# Autodesk Inventor assembly: Joint2
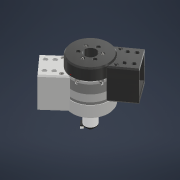
[picture p0: Inventor's stored thumbnail of the model, 180x180]
Saved by Autodesk Inventor 2021 (Build 250183000, 183)
## iProperties
RuleStatus: InUse
Created: 2025-03-14
Part Number: Joint2
Document SubType Name: Assembly
Designer: rocke
Mass: 414.793 g
Surface Area: 1158.92 cm^2
Volume: 253.092 cm^3
Density: 1.6389 g/cm^3
Author: rocke
## Documents named in this file (26)
- C:\Users\rocke\Documents\Robot Arm IPT\Joint2.iam
- C:\Users\rocke\Documents\Robot Arm IPT\Joint2\Design Accelerator\Spur Gears1.iam
- C:\Users\rocke\Documents\Robot Arm IPT\Joint2\Design Accelerator\Spur Gears3.iam
- C:\Users\rocke\Documents\Inventor\Content Center Files\R2021\en-US\DIN 472(2)\DIN 472 - 16x1.ipt
- C:\Users\rocke\Documents\Inventor\Content Center Files\R2021\en-US\DIN 625 SKF(4)\DIN 625 SKF - SKF 628_8-2Z.ipt
- C:\Users\rocke\Downloads\12V 350RPM Small DFRobot Motor v8.iam
- C:\Users\rocke\Documents\Inventor\Content Center Files\R2021\en-US\ISO 4762(2)\ISO 4762 - M3 x 5ISO.ipt
- C:\Users\rocke\Documents\Robot Arm IPT\Joint2\Design Accelerator\Spur Gear11.ipt
- C:\Users\rocke\Documents\Inventor\Content Center Files\R2021\en-US\GB_T 276-94 60000-2Z\Bearing 61809-2Z GB_T 276-94.ipt
- C:\Users\rocke\Documents\Robot Arm IPT\Joint2\Planet Subassembly.iam
- C:\Users\rocke\Downloads\TO-92 flat Formed Leads Horizontal Back.ipt
- C:\Users\rocke\Documents\Inventor\Content Center Files\R2021\en-US\ANSI B 18.2.4.1 M(1)\ANSI B 18.2.4.1 M - M3 x 0.5Style 1.ipt
- C:\Users\rocke\Documents\Inventor\Content Center Files\R2021\en-US\ISO 4026\ISO 4026 - M3 x 8 - ISO.ipt
- C:\Users\rocke\Documents\Inventor\Content Center Files\R2021\en-US\ANSI B18.3.1M(1)\ANSI B18.3.1M - M3x0.5 x 60(2).ipt
- C:\Users\rocke\Documents\Inventor\Content Center Files\R2021\en-US\DIN 985\DIN 985 - M3.ipt
- C:\Users\rocke\Documents\Inventor\Content Center Files\R2021\en-US\ISO 4032(2)\ISO 4032 - M4 - ISO.ipt
- C:\Users\rocke\Documents\Inventor\Content Center Files\R2021\en-US\ANSI B18.3.1M(1)\ANSI B18.3.1M - M4x0.7 x 60(2).ipt
- C:\Users\rocke\Documents\Inventor\Content Center Files\R2021\en-US\ANSI B18.3.1M(1)\ANSI B18.3.1M - M4x0.7 x 65(2).ipt
- C:\Users\rocke\Documents\Robot Arm IPT\Moving Link Fixation\Moving_Link_Fixation.iam
- C:\Users\rocke\Documents\Robot Arm IPT\Fixed Link Fixation\Fixed_Link_Fixation.iam
- C:\Users\rocke\Documents\Robot Arm IPT\Ring Gear 1\Ring_Gear_Assembly_1.iam
- C:\Users\rocke\Documents\Robot Arm IPT\Planet Carrier\Planet_Carrier_Bottom.ipt
- C:\Users\rocke\Documents\Robot Arm IPT\Planet Carrier\Planet_Carrier_Mid.ipt
- C:\Users\rocke\Documents\Robot Arm IPT\Planet Carrier\Planet_Carrier_Top.ipt
- C:\Users\rocke\Documents\Robot Arm IPT\Ring Cover\Ring_Cover_Bot.ipt
- C:\Users\rocke\Documents\Robot Arm IPT\Ring Cover\Ring_Cover_Top.ipt
## Components (44 placed, 24 different names)
1. Spur Gears:1 [sub-assembly]
2. Spur Gears:2 [sub-assembly] — Rigid:9, Rigid:13, Mate:16
3. Planet_Carrier_Bottom:1 — Rotational:3, Rotational:4, Rotational:5, Rigid:2, Rigid:4
4. Planet_Carrier_Mid:1 — Rigid:4, Rigid:5, Rigid:8
5. Planet_Carrier_Top:1 — Rigid:5, Rigid:7, Rigid:15
6. Ring_Cover_Bot:1 — Rotational:1, Mate:1, Mate:2, Mate:3, Mate:4, Mate:5, Rigid:9, Insert:2
7. Sun_Gear — Rotational:2, Rigid:1, Insert:1
8. Ring_Cover_Top:1 — Rotational:6, Rigid:13, Rigid:14, Mate:42, Mate:46, Mate:50, Mate:54, Mate:58
9. Ring_Gear_Assembly_1:1 [sub-assembly] — Rotational:3, Mate:6, Mate:7
10. Planet Subassembly:2 [sub-assembly] — Rotational:5, Mate:10, Mate:11
11. Planet Subassembly:3 [sub-assembly] — Rotational:4, Mate:14, Mate:15
12. Fixed_Link_Fixation:1 [sub-assembly] — Insert:2, Mate:16, Mate:29, Mate:30, Mate:39, Mate:40, Mate:41, Mate:43, Mate:44, Mate:45, Mate:47, Mate:48, Mate:49, Mate:51, Mate:52, Mate:53, Mate:55, Mate:56, Mate:57, Mate:63, Mate:64, Mate:65, Mate:66, Mate:67, Mate:68, Mate:69, Mate:70
13. Moving_Link_Fixation:1 [sub-assembly] — Rigid:10, Rigid:11, Rigid:12, Rigid:15
14. DIN 472 16x1:1 — Rigid:2, Rigid:3
15. Broached Socket Head Cap Screw - Metric M4x0.7 x 60:6 — Mate:55, Mate:56
16. ISO 4032 M4:1 — Mate:57, Mate:58
17. Broached Socket Head Cap Screw - Metric M4x0.7 x 60:3 — Mate:43, Mate:44
18. ISO 4032 M4:2 — Mate:45, Mate:46
19. Broached Socket Head Cap Screw - Metric M4x0.7 x 60:5 — Mate:51, Mate:52
20. ISO 4032 M4:3 — Mate:53, Mate:54
21. Broached Socket Head Cap Screw - Metric M4x0.7 x 60:1 — Mate:29, Mate:30
22. Broached Socket Head Cap Screw - Metric M4x0.7 x 60:2 — Mate:39, Mate:40
23. ISO 4032 M4:4 — Mate:41, Mate:42
24. Broached Socket Head Cap Screw - Metric M4x0.7 x 60:4 — Mate:47, Mate:48
25. ISO 4032 M4:5 — Mate:49, Mate:50
26. Broached Socket Head Cap Screw - Metric M4x0.7 x 65:2 — Mate:67, Mate:68
27. ISO 4032 M4:6 — Mate:69, Mate:70
28. Broached Socket Head Cap Screw - Metric M4x0.7 x 65:1 — Mate:63, Mate:64
29. ISO 4032 M4:7 — Mate:65, Mate:66
30. Broached Socket Head Cap Screw - Metric M3x0.5 x 60:1 — Mate:6, Mate:7
31. DIN 985 - replaced by DIN EN ISO 10511 M3:1 — Rigid:12
32. Broached Socket Head Cap Screw - Metric M3x0.5 x 60:2 — Mate:10, Mate:11
33. DIN 985 - replaced by DIN EN ISO 10511 M3:2 — Rigid:11
34. Broached Socket Head Cap Screw - Metric M3x0.5 x 60:3 — Mate:14, Mate:15
35. DIN 985 - replaced by DIN EN ISO 10511 M3:3 — Rigid:10
36. Hex Nut Metric M3 x 0.5:1 — Rotational:2
37. ISO 4026 M3 x 8:1 — Rigid:1
38. ISO 4762 M3 x 5:1 — Mate:2, Mate:3
39. ISO 4762 M3 x 5:2 — Mate:4, Mate:5
40. DIN 625 SKF- with two Z shields SKF 628/8-2Z:1 — Rigid:3
41. Rolling bearing GB/T 276-1994 Type 60000-2Z 61809-2Z:1 — Rigid:7, Rotational:6
42. Rolling bearing GB/T 276-1994 Type 60000-2Z 61809-2Z:2 — Rigid:8
43. 12V 350RPM Small DFRobot Motor v8:1 [sub-assembly] — Rotational:1, Mate:1, Insert:1
44. TO-92 flat Formed Leads Horizontal Back:1 — Rigid:14
## Relationships (64: Mate 42, WeldJoint 14, RevoluteJoint 6, Insert 2)
- Rotational:1 [RevoluteJoint]: Ring_Cover_Bot:1 ↔ 12V 350RPM Small DFRobot Motor v8:1
- Mate:1: Ring_Cover_Bot:1 ↔ 12V 350RPM Small DFRobot Motor v8:1
- Mate:2: Ring_Cover_Bot:1 ↔ ISO 4762 M3 x 5:1
- Mate:3: Ring_Cover_Bot:1 ↔ ISO 4762 M3 x 5:1
- Mate:4: Ring_Cover_Bot:1 ↔ ISO 4762 M3 x 5:2
- Mate:5: Ring_Cover_Bot:1 ↔ ISO 4762 M3 x 5:2
- Rotational:2 [RevoluteJoint]: Sun_Gear ↔ Hex Nut Metric M3 x 0.5:1
- Rigid:1 [WeldJoint]: Sun_Gear ↔ ISO 4026 M3 x 8:1
- Insert:1: Sun_Gear ↔ 12V 350RPM Small DFRobot Motor v8:1
- Rotational:3 [RevoluteJoint]: Planet_Carrier_Bottom:1 ↔ Ring_Gear_Assembly_1:1
- Rotational:4 [RevoluteJoint]: Planet_Carrier_Bottom:1 ↔ Planet Subassembly:3
- Rotational:5 [RevoluteJoint]: Planet_Carrier_Bottom:1 ↔ Planet Subassembly:2
- Rigid:2 [WeldJoint]: Planet_Carrier_Bottom:1 ↔ DIN 472 16x1:1
- Rigid:3 [WeldJoint]: DIN 472 16x1:1 ↔ DIN 625 SKF- with two Z shields SKF 628/8-2Z:1
- Rigid:4 [WeldJoint]: Planet_Carrier_Bottom:1 ↔ Planet_Carrier_Mid:1
- Rigid:5 [WeldJoint]: Planet_Carrier_Mid:1 ↔ Planet_Carrier_Top:1
- Mate:6: Ring_Gear_Assembly_1:1 ↔ Broached Socket Head Cap Screw - Metric M3x0.5 x 60:1
- Mate:7: Ring_Gear_Assembly_1:1 ↔ Broached Socket Head Cap Screw - Metric M3x0.5 x 60:1
- Mate:10: Planet Subassembly:2 ↔ Broached Socket Head Cap Screw - Metric M3x0.5 x 60:2
- Mate:11: Planet Subassembly:2 ↔ Broached Socket Head Cap Screw - Metric M3x0.5 x 60:2
- Mate:14: Planet Subassembly:3 ↔ Broached Socket Head Cap Screw - Metric M3x0.5 x 60:3
- Mate:15: Planet Subassembly:3 ↔ Broached Socket Head Cap Screw - Metric M3x0.5 x 60:3
- Rigid:7 [WeldJoint]: Planet_Carrier_Top:1 ↔ Rolling bearing GB/T 276-1994 Type 60000-2Z 61809-2Z:1
- Rigid:8 [WeldJoint]: Planet_Carrier_Mid:1 ↔ Rolling bearing GB/T 276-1994 Type 60000-2Z 61809-2Z:2
- Rotational:6 [RevoluteJoint]: Ring_Cover_Top:1 ↔ Rolling bearing GB/T 276-1994 Type 60000-2Z 61809-2Z:1
- Rigid:9 [WeldJoint]: Spur Gears:2 ↔ Ring_Cover_Bot:1
- Rigid:10 [WeldJoint]: Moving_Link_Fixation:1 ↔ DIN 985 - replaced by DIN EN ISO 10511 M3:3
- Rigid:11 [WeldJoint]: Moving_Link_Fixation:1 ↔ DIN 985 - replaced by DIN EN ISO 10511 M3:2
- Rigid:12 [WeldJoint]: Moving_Link_Fixation:1 ↔ DIN 985 - replaced by DIN EN ISO 10511 M3:1
- Rigid:13 [WeldJoint]: Spur Gears:2 ↔ Ring_Cover_Top:1
- Rigid:14 [WeldJoint]: Ring_Cover_Top:1 ↔ TO-92 flat Formed Leads Horizontal Back:1
- Rigid:15 [WeldJoint]: Planet_Carrier_Top:1 ↔ Moving_Link_Fixation:1
- Insert:2: Ring_Cover_Bot:1 ↔ Fixed_Link_Fixation:1
- Mate:16: Spur Gears:2 ↔ Fixed_Link_Fixation:1
- Mate:29: Fixed_Link_Fixation:1 ↔ Broached Socket Head Cap Screw - Metric M4x0.7 x 60:1
- Mate:30: Fixed_Link_Fixation:1 ↔ Broached Socket Head Cap Screw - Metric M4x0.7 x 60:1
- Mate:39: Fixed_Link_Fixation:1 ↔ Broached Socket Head Cap Screw - Metric M4x0.7 x 60:2
- Mate:40: Fixed_Link_Fixation:1 ↔ Broached Socket Head Cap Screw - Metric M4x0.7 x 60:2
- Mate:41: Fixed_Link_Fixation:1 ↔ ISO 4032 M4:4
- Mate:42: Ring_Cover_Top:1 ↔ ISO 4032 M4:4
- Mate:43: Fixed_Link_Fixation:1 ↔ Broached Socket Head Cap Screw - Metric M4x0.7 x 60:3
- Mate:44: Fixed_Link_Fixation:1 ↔ Broached Socket Head Cap Screw - Metric M4x0.7 x 60:3
- Mate:45: Fixed_Link_Fixation:1 ↔ ISO 4032 M4:2
- Mate:46: Ring_Cover_Top:1 ↔ ISO 4032 M4:2
- Mate:47: Fixed_Link_Fixation:1 ↔ Broached Socket Head Cap Screw - Metric M4x0.7 x 60:4
- Mate:48: Fixed_Link_Fixation:1 ↔ Broached Socket Head Cap Screw - Metric M4x0.7 x 60:4
- Mate:49: Fixed_Link_Fixation:1 ↔ ISO 4032 M4:5
- Mate:50: Ring_Cover_Top:1 ↔ ISO 4032 M4:5
- Mate:51: Fixed_Link_Fixation:1 ↔ Broached Socket Head Cap Screw - Metric M4x0.7 x 60:5
- Mate:52: Fixed_Link_Fixation:1 ↔ Broached Socket Head Cap Screw - Metric M4x0.7 x 60:5
- Mate:53: Fixed_Link_Fixation:1 ↔ ISO 4032 M4:3
- Mate:54: Ring_Cover_Top:1 ↔ ISO 4032 M4:3
- Mate:55: Fixed_Link_Fixation:1 ↔ Broached Socket Head Cap Screw - Metric M4x0.7 x 60:6
- Mate:56: Fixed_Link_Fixation:1 ↔ Broached Socket Head Cap Screw - Metric M4x0.7 x 60:6
- Mate:57: Fixed_Link_Fixation:1 ↔ ISO 4032 M4:1
- Mate:58: Ring_Cover_Top:1 ↔ ISO 4032 M4:1
- Mate:63: Fixed_Link_Fixation:1 ↔ Broached Socket Head Cap Screw - Metric M4x0.7 x 65:1
- Mate:64: Fixed_Link_Fixation:1 ↔ Broached Socket Head Cap Screw - Metric M4x0.7 x 65:1
- Mate:65: Fixed_Link_Fixation:1 ↔ ISO 4032 M4:7
- Mate:66: Fixed_Link_Fixation:1 ↔ ISO 4032 M4:7
- Mate:67: Fixed_Link_Fixation:1 ↔ Broached Socket Head Cap Screw - Metric M4x0.7 x 65:2
- Mate:68: Fixed_Link_Fixation:1 ↔ Broached Socket Head Cap Screw - Metric M4x0.7 x 65:2
- Mate:69: Fixed_Link_Fixation:1 ↔ ISO 4032 M4:6
- Mate:70: Fixed_Link_Fixation:1 ↔ ISO 4032 M4:6
